# Autodesk Inventor assembly: Link3
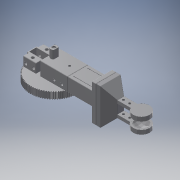
[picture p0: Inventor's stored thumbnail of the model, 180x180]
Saved by Autodesk Inventor 2019 (Build 230136000, 136)
## iProperties
Created: 2020-02-16
Part Number: Link3
Document SubType Name: Assembly
Designer: Alex
Author: Alex
## Documents named in this file (7)
- D:\Alex\Documents\GitHub\RBE3001-URDF-Example\STLs\FinalSTLS\Inventor_Assy\Link3.iam
- D:\Alex\Documents\Personal Projects\BenchPowerSupply\Link3_Cup2.ipt
- D:\Alex\Documents\Personal Projects\BenchPowerSupply\Link3_DrivenGear.ipt
- D:\Alex\Documents\Personal Projects\BenchPowerSupply\Link3_Frame.ipt
- D:\Alex\Documents\Personal Projects\BenchPowerSupply\Link3_LoadCellBlock.ipt
- D:\Alex\Documents\Personal Projects\BenchPowerSupply\Link3_Cup1.ipt
- D:\Alex\Documents\GitHub\RBE3001-URDF-Example\STLs\FinalSTLS\Inventor_Assy\Gripper_LowRes.ipt
## Components (6 placed, 6 different names)
1. Link3_Frame:1 — Flush:7, Flush:8, Flush:9, Mate:1, Flush:16, Flush:17
2. Link3_LoadCellBlock:1 — Flush:10, Flush:11, Flush:12
3. Link3_Cup1:1 — Flush:13, Flush:14, Flush:15
4. Link3_Cup2:1 — Flush:1, Flush:2, Flush:3
5. Link3_DrivenGear:1 — Flush:4, Flush:5, Flush:6
6. Gripper_LowRes:1 — Mate:1, Flush:16, Flush:17
## Relationships (18: Flush 17, Mate 1)
- Flush:1: Link3_Cup2:1
- Flush:2: Link3_Cup2:1
- Flush:3: Link3_Cup2:1
- Flush:4: Link3_DrivenGear:1
- Flush:5: Link3_DrivenGear:1
- Flush:6: Link3_DrivenGear:1
- Flush:7: Link3_Frame:1
- Flush:8: Link3_Frame:1
- Flush:9: Link3_Frame:1
- Flush:10: Link3_LoadCellBlock:1
- Flush:11: Link3_LoadCellBlock:1
- Flush:12: Link3_LoadCellBlock:1
- Flush:13: Link3_Cup1:1
- Flush:14: Link3_Cup1:1
- Flush:15: Link3_Cup1:1
- Mate:1: Link3_Frame:1 ↔ Gripper_LowRes:1
- Flush:16: Link3_Frame:1 ↔ Gripper_LowRes:1
- Flush:17: Link3_Frame:1 ↔ Gripper_LowRes:1
